# Autodesk Inventor assembly: BodyCasing
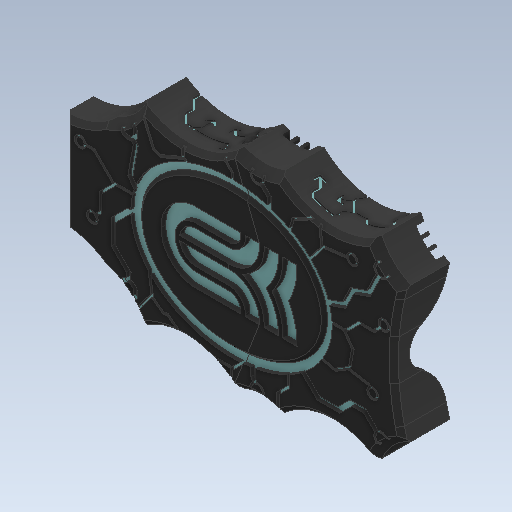
[picture p0: Inventor's stored thumbnail of the model, 512x512]
Saved by Autodesk Inventor 2020 (Build 240168000, 168)
## iProperties
Created: 2021-03-18
Part Number: BodyCasing
Document SubType Name: Assembly
Designer: Turing
Author: Turing
## Documents named in this file (3)
- D:\HexapodFinal v3\BodyCasing.iam
- D:\HexapodFinal v3\BodyTopCasing2.ipt
- D:\HexapodFinal v3\BodyTopCasing1.ipt
## Components (2 placed, 2 different names)
1. BodyTopCasing2:1 — Rigid:1
2. BodyTopCasing1:1 — Rigid:1
## Relationships (1: WeldJoint 1)
- Rigid:1 [WeldJoint]: BodyTopCasing2:1 ↔ BodyTopCasing1:1
